# Autodesk Inventor assembly: completed project
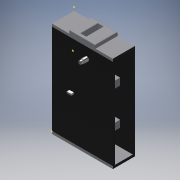
[picture p0: Inventor's stored thumbnail of the model, 180x180]
Saved by Autodesk Inventor 2019 (Build 230136000, 136)
## iProperties
Created: 2020-02-19
Part Number: completed project
Document SubType Name: Assembly
Designer: LENOVO
Author: LENOVO
## Documents named in this file (8)
- C:\Users\LENOVO\Desktop\fouzan\completed project.iam
- C:\Users\LENOVO\Desktop\fouzan\back plate.ipt
- C:\Users\LENOVO\Desktop\fouzan\closing.ipt
- C:\Users\LENOVO\Desktop\fouzan\dc motor.ipt
- C:\Users\LENOVO\Desktop\fouzan\bear.ipt
- C:\Users\LENOVO\Desktop\fouzan\roller of 4 cm.ipt
- C:\Users\LENOVO\Desktop\fouzan\servo part.ipt
- C:\Users\LENOVO\Desktop\fouzan\servo part1.ipt
## Components (10 placed, 7 different names)
1. back plate:1 — Mate:1, Mate:2, Mate:3, Mate:5, Mate:6, Rigid:1, Rigid:2, Mate:8, Mate:9, Mate:10
2. closing:1 — Mate:2, Mate:10, Mate:11, Mate:12, Mate:13, Mate:14
3. dc motor:1 — Mate:1, Mate:4, Mate:5
4. bear:1 — Mate:3, Mate:6, Mate:7
5. roller of 4 cm:1 — Mate:7, Rigid:1
6. roller of 4 cm:2 — Mate:4, Rigid:2
7. servo part:1 — Mate:8, Mate:9, Mate:15, Rigid:3
8. bear:2 — Mate:11, Mate:13
9. bear:3 — Mate:12, Mate:14
10. servo part1:1 — Mate:15, Rigid:3
## Relationships (18: Mate 15, WeldJoint 3)
- Mate:1: back plate:1 ↔ dc motor:1
- Mate:2: back plate:1 ↔ closing:1
- Mate:3: back plate:1 ↔ bear:1
- Mate:4: dc motor:1 ↔ roller of 4 cm:2
- Mate:5: back plate:1 ↔ dc motor:1
- Mate:6: back plate:1 ↔ bear:1
- Mate:7: bear:1 ↔ roller of 4 cm:1
- Rigid:1 [WeldJoint] (-53.34 mm): back plate:1 ↔ roller of 4 cm:1
- Rigid:2 [WeldJoint] (55.88 mm): back plate:1 ↔ roller of 4 cm:2
- Mate:8: back plate:1 ↔ servo part:1
- Mate:9: back plate:1 ↔ servo part:1
- Mate:10: back plate:1 ↔ closing:1
- Mate:11: closing:1 ↔ bear:2
- Mate:12: closing:1 ↔ bear:3
- Mate:13: closing:1 ↔ bear:2
- Mate:14: closing:1 ↔ bear:3
- Mate:15: servo part:1 ↔ servo part1:1
- Rigid:3 [WeldJoint] (-2.54 mm): servo part:1 ↔ servo part1:1
